# Autodesk Inventor assembly: Z-head-assembly-IKO-T1-NEMA8
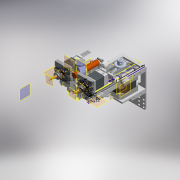
[picture p0: Inventor's stored thumbnail of the model, 180x180]
Saved by Autodesk Inventor 2016 (Build 200138000, 138)
## iProperties
Created: 2015-05-08
Part Number: Z-head-assembly-IKO-T1-NEMA8
Document SubType Name: Assembly
Designer: ax
Mass: 653.738 g
Surface Area: 1248.62 cm^2
Volume: 178.22 cm^3
Density: 3.66816 g/cm^3
Author: ax
## Documents named in this file (34)
- C:\Users\as\Documents\Inventor\mintplacer-export\Z-head-assembly-IKO-T1-NEMA8.iam
- C:\Users\as\Documents\Inventor\mintplacer-export\Z-head-baseplate-IKO.ipt
- C:\Users\as\Documents\Inventor\mintplacer-export\BSPG15_60__40_.iam
- C:\Users\as\Documents\Inventor\mintplacer-export\C-head-base.ipt
- C:\Users\as\Documents\Inventor\mintplacer-export\C-head-side.ipt
- C:\Users\as\Documents\Inventor\mintplacer-export\GT2_20tooth.ipt
- C:\Users\as\Documents\Inventor\mintplacer-export\GT2-belt-2MR-200-06.ipt
- C:\Users\as\Documents\Inventor\mintplacer-export\HTD-5M-belt-clamp.ipt
- C:\Users\as\Documents\Inventor\mintplacer-export\GT2 belt clamp.ipt
- C:\Users\as\Documents\Inventor\mintplacer-export\nozzle-assembly.iam
- C:\Users\as\Documents\Inventor\mintplacer-export\Nanotec-ST4118S1404.iam
- C:\Users\as\Documents\Inventor\mintplacer-export\c-head-flange.ipt
- C:\Users\as\Documents\Inventor\mintplacer-export\Z-head-assembly-IKO-T1\Design Accelerator\Bolted Connection3.iam
- C:\Users\as\Documents\Inventor\mintplacer-export\Z-head-assembly-IKO-T1\Design Accelerator\Bolted Connection4.iam
- C:\Users\as\Documents\Inventor\mintplacer-export\Z-head-assembly-IKO-T1\Design Accelerator\Bolted Connection5.iam
- C:\Users\as\Documents\Inventor\mintplacer-export\Z-head-assembly-IKO-T1\Design Accelerator\Bolted Connection6.iam
- C:\Users\as\Documents\Inventor\mintplacer-export\Z-head-assembly-IKO-T1\Design Accelerator\Bolted Connection7.iam
- C:\Users\as\Documents\Inventor\mintplacer-export\small-tact-switch.ipt
- C:\Users\as\Documents\Inventor\mintplacer-export\Z-head-assembly-IKO-T1\Design Accelerator\Bolted Connection8.iam
- C:\Users\as\Documents\Inventor\mintplacer-export\Z-head-assembly-IKO-T1\Design Accelerator\Bolted Connection9.iam
- C:\Users\as\Documents\Inventor\mintplacer-export\Z-head-assembly-IKO-T1\Design Accelerator\Bolted Connection10.iam
- C:\Users\as\Documents\Inventor\mintplacer-export\Z-head-assembly-IKO-T1\Design Accelerator\Bolted Connection11.iam
- C:\Users\as\Documents\Inventor\Content Center Files\R2016\en-US\ISO 4762(1)\DIN EN ISO 4762 - M3 x 12.ipt
- C:\Users\as\Documents\Inventor\mintplacer-export\render\cam-flying.iam
- C:\Users\as\Documents\Inventor\mintplacer-export\Z-head-assembly-IKO-T1\Design Accelerator\Bolted Connection13.iam
- C:\Users\as\Documents\Inventor\mintplacer-export\Z-head-assembly-IKO-T1\Design Accelerator\Bolted Connection14.iam
- C:\Users\as\Documents\Inventor\mintplacer-export\render\Z-head-sideplate.ipt
- C:\Users\as\Documents\Inventor\mintplacer-export\Z-head-topplate.ipt
- C:\Users\as\Documents\Inventor\mintplacer-export\render\Z-head-beltmount.ipt
- C:\Users\as\Documents\Inventor\mintplacer-export\Z-head-assembly-IKO-T1\Design Accelerator\Bolted Connection15.iam
- C:\Users\as\Documents\Inventor\mintplacer-export\Z-head-assembly-IKO-T1\Design Accelerator\Bolted Connection16.iam
- C:\Users\as\Documents\Inventor\mintplacer-export\Z-head-assembly-IKO-T1\Design Accelerator\Bolted Connection17.iam
- C:\Users\as\Documents\Inventor\mintplacer-export\Z-head-assembly-IKO-T1\Design Accelerator\Bolted Connection18.iam
- C:\Users\as\Documents\Inventor\mintplacer-export\Nanotec-NEMA8-st2018s0604\st2018s0604.iam
## Components (69 placed, 19 different names)
1. Z-head-baseplate-IKO:1 — Mate:1, Flush:1, Flush:7, Mate:5, Mate:10, Mate:39, Mate:40, Mate:41, Mate:70, Mate:71, Mate:74, Mate:76, Mate:110, Flush:31, Mate:111, Mate:112, Mate:116, Angle:1, Mate:118, Flush:36, Flush:37, Flush:38, Mate:121, Mate:133, Mate:135, Flush:43, Flush:44
2. HTD-5M-belt-clamp:1 — Mate:131, Flush:42
3. Nanotec-ST4118S1404:2 [sub-assembly] — Mate:5, Mate:10, Cylindrical:1, Mate:72, Mate:73, Mate:75, Flush:33, Mate:117
4. GT2_20tooth:1 — Mate:4, Cylindrical:1
5. BSPG15_60__40_:1 [sub-assembly] — Mate:1, Flush:1, Flush:3, Mate:11, Flush:19, Flush:20, Mate:84, Mate:86, Mate:122, Flush:44
6. c-head-flange:1 — Flush:14, Flush:15, Mate:11, Mate:12, Flush:17, Flush:19, Mate:32, Mate:33, Mate:34, Flush:20, Mate:83, Mate:85, Mate:87, Mate:88, Mate:130
7. C-head-base:1 — Flush:3, Flush:13, Flush:14, Flush:15, Flush:18, Mate:17, Mate:78, Mate:142, Mate:143
8. C-head-side:1 — Mate:7, Flush:11, Flush:13, Mate:12, Flush:17, Flush:18, Mate:17, Mate:77, Flush:34, Mate:129
9. st2018s0604:1 [sub-assembly] — Mate:142, Mate:143, Mate:144
10. nozzle-assembly:1 [sub-assembly] — Mate:144
11. GT2 belt clamp:1 — Mate:7, Flush:11, Flush:34, Mate:127, Mate:128
12. Bolted Connection:3 [sub-assembly] — Mate:77, Mate:78
13. Bolted Connection:4 [sub-assembly] — Mate:129, Mate:130
14. Bolted Connection:5 [sub-assembly] — Mate:127, Mate:128
15. Bolted Connection:6 [sub-assembly] — Mate:83, Mate:84
16. Bolted Connection:7 [sub-assembly] — Mate:85, Mate:86
17. small-tact-switch:1 — Mate:32, Mate:33, Mate:34, Mate:89, Mate:90
18. Bolted Connection:8 [sub-assembly] — Mate:87, Mate:88
19. small-tact-switch:2 — Mate:123, Mate:124
20. small-tact-switch:3 — Mate:39, Mate:40, Mate:41, Mate:125, Mate:126
21. Bolted Connection:9 [sub-assembly] — Mate:89, Mate:90
22. Bolted Connection:10 [sub-assembly] — Mate:125, Mate:126
23. Bolted Connection:12 [sub-assembly] — Mate:123, Mate:124
24. DIN EN ISO 4762 M3 x 12:1 — Mate:70, Mate:117
25. DIN EN ISO 4762 M3 x 12:2 — Mate:71, Mate:72
26. DIN EN ISO 4762 M3 x 12:3 — Mate:74, Mate:75
27. DIN EN ISO 4762 M3 x 12:4 — Mate:73, Mate:76
28. cam-flying:1 [sub-assembly] — Mate:110, Flush:31, Mate:111, Mate:113
29. Bolted Connection:13 [sub-assembly] — Mate:112, Mate:113
30. Bolted Connection:14 [sub-assembly] — Mate:121, Mate:122
31. Z-head-sideplate:1 — Mate:119, Flush:39, Flush:40, Mate:120, Mate:134, Mate:138
32. Z-head-topplate:1 — Flush:36, Flush:37, Flush:38, Mate:119, Flush:39, Flush:40, Flush:41, Mate:132, Mate:140
33. Z-head-beltmount:1 — Flush:41, Mate:120, Mate:131, Flush:42, Flush:43, Mate:139, Mate:141
34. Bolted Connection:15 [sub-assembly] — Mate:132, Mate:133
35. Bolted Connection:16 [sub-assembly] — Mate:134, Mate:135
36. Bolted Connection:17 [sub-assembly] — Mate:140, Mate:141
37. Bolted Connection:18 [sub-assembly] — Mate:138, Mate:139
38. BSPG15_60__40_:2 [sub-assembly] — Flush:45, Flush:50, Flush:51, Mate:148, Mate:153, Mate:155, Mate:162
39. C-head-base:2 — Flush:45, Flush:46, Mate:145, Flush:47, Flush:53, Flush:54, Mate:149, Mate:164, Mate:165
40. C-head-side:2 — Flush:46, Mate:145, Flush:47, Mate:146, Flush:48, Flush:49, Flush:52, Mate:147, Flush:55, Flush:56
41. GT2 belt clamp:2 — Mate:146, Flush:48, Flush:49, Mate:151, Mate:152
42. nozzle-assembly:2 [sub-assembly] — Mate:163
43. c-head-flange:2 — Flush:50, Flush:51, Flush:52, Mate:147, Mate:148, Flush:53, Flush:54, Mate:150, Mate:154, Mate:156, Mate:157, Mate:158, Flush:57, Mate:159, Mate:160
44. Bolted Connection:19 [sub-assembly] — Mate:149, Flush:55
45. Bolted Connection:20 [sub-assembly] — Mate:150, Flush:56
46. Bolted Connection:21 [sub-assembly] — Mate:151, Mate:152
47. Bolted Connection:22 [sub-assembly] — Mate:153, Mate:154
48. Bolted Connection:23 [sub-assembly] — Mate:155, Mate:156
49. small-tact-switch:4 — Mate:157, Mate:158, Flush:57, Mate:161, Flush:58
50. Bolted Connection:24 [sub-assembly] — Mate:159, Mate:160
51. Bolted Connection:25 [sub-assembly] — Mate:161, Flush:58
52. Bolted Connection:26 [sub-assembly] — Mate:162
53. st2018s0604:2 [sub-assembly] — Mate:163, Mate:164, Mate:165
54. GT2-belt-2MR-200-06:1 — Mate:4, Mate:118
55. GT2-belt-2MR-200-06:2
56. GT2-belt-2MR-200-06:3
57. GT2-belt-2MR-200-06:4
58. GT2-belt-2MR-200-06:5
59. GT2-belt-2MR-200-06:6
60. GT2-belt-2MR-200-06:7
61. GT2-belt-2MR-200-06:8
62. GT2-belt-2MR-200-06:9
63. GT2-belt-2MR-200-06:10
64. GT2-belt-2MR-200-06:11
65. GT2-belt-2MR-200-06:12
66. GT2-belt-2MR-200-06:13
67. GT2-belt-2MR-200-06:14
68. GT2-belt-2MR-200-06:15
69. GT2-belt-2MR-200-06:16
## Component patterns: (8 elements, first: GT2-belt-2MR-200-06:1), (8 elements, first: GT2-belt-2MR-200-06:9)
## Relationships (124: Mate 83, Flush 39, CylindricalJoint 1, Angle 1)
- Mate:1: Z-head-baseplate-IKO:1 ↔ BSPG15_60__40_:1
- Flush:1: Z-head-baseplate-IKO:1 ↔ BSPG15_60__40_:1
- Flush:3: BSPG15_60__40_:1 ↔ C-head-base:1
- Mate:4 (1 mm): GT2_20tooth:1 ↔ GT2-belt-2MR-200-06:1
- Flush:7 (-6.3662 mm): Z-head-baseplate-IKO:1
- Mate:5 (-21 mm): Z-head-baseplate-IKO:1 ↔ Nanotec-ST4118S1404:2
- Flush:8 (-1.15 mm)
- Mate:7: C-head-side:1 ↔ GT2 belt clamp:1
- Flush:11: C-head-side:1 ↔ GT2 belt clamp:1
- Flush:13: C-head-base:1 ↔ C-head-side:1
- Mate:10: Z-head-baseplate-IKO:1 ↔ Nanotec-ST4118S1404:2
- Cylindrical:1: Nanotec-ST4118S1404:2 ↔ GT2_20tooth:1
- Flush:14: c-head-flange:1 ↔ C-head-base:1
- Flush:15: c-head-flange:1 ↔ C-head-base:1
- Mate:11: BSPG15_60__40_:1 ↔ c-head-flange:1
- Mate:12: c-head-flange:1 ↔ C-head-side:1
- Flush:17: c-head-flange:1 ↔ C-head-side:1
- Flush:18: C-head-base:1 ↔ C-head-side:1
- Flush:19: BSPG15_60__40_:1 ↔ c-head-flange:1
- Mate:17: C-head-base:1 ↔ C-head-side:1
- Mate:32: c-head-flange:1 ↔ small-tact-switch:1
- Mate:33: c-head-flange:1 ↔ small-tact-switch:1
- Mate:34: c-head-flange:1 ↔ small-tact-switch:1
- Flush:20: BSPG15_60__40_:1 ↔ c-head-flange:1
- Mate:39: Z-head-baseplate-IKO:1 ↔ small-tact-switch:3
- Mate:40: Z-head-baseplate-IKO:1 ↔ small-tact-switch:3
- Mate:41: Z-head-baseplate-IKO:1 ↔ small-tact-switch:3
- Mate:70: Z-head-baseplate-IKO:1 ↔ DIN EN ISO 4762 M3 x 12:1
- Mate:71: Z-head-baseplate-IKO:1 ↔ DIN EN ISO 4762 M3 x 12:2
- Mate:72: Nanotec-ST4118S1404:2 ↔ DIN EN ISO 4762 M3 x 12:2
- Mate:73: Nanotec-ST4118S1404:2 ↔ DIN EN ISO 4762 M3 x 12:4
- Mate:74: Z-head-baseplate-IKO:1 ↔ DIN EN ISO 4762 M3 x 12:3
- Mate:75: Nanotec-ST4118S1404:2 ↔ DIN EN ISO 4762 M3 x 12:3
- Mate:76: Z-head-baseplate-IKO:1 ↔ DIN EN ISO 4762 M3 x 12:4
- Mate:77: C-head-side:1 ↔ Bolted Connection:3
- Mate:78: C-head-base:1 ↔ Bolted Connection:3
- Mate:83: c-head-flange:1 ↔ Bolted Connection:6
- Mate:84: BSPG15_60__40_:1 ↔ Bolted Connection:6
- Mate:85: c-head-flange:1 ↔ Bolted Connection:7
- Mate:86: BSPG15_60__40_:1 ↔ Bolted Connection:7
- Mate:87: c-head-flange:1 ↔ Bolted Connection:8
- Mate:88: c-head-flange:1 ↔ Bolted Connection:8
- Mate:89: small-tact-switch:1 ↔ Bolted Connection:9
- Mate:90: small-tact-switch:1 ↔ Bolted Connection:9
- Mate:110: Z-head-baseplate-IKO:1 ↔ cam-flying:1
- Flush:31: Z-head-baseplate-IKO:1 ↔ cam-flying:1
- Mate:111: Z-head-baseplate-IKO:1 ↔ cam-flying:1
- Mate:112: Z-head-baseplate-IKO:1 ↔ Bolted Connection:13
- Mate:113: cam-flying:1 ↔ Bolted Connection:13
- Mate:116: Z-head-baseplate-IKO:1
- Angle:1 (0 deg): Z-head-baseplate-IKO:1
- Flush:32 (-79 mm)
- Flush:33 (-21 mm): Nanotec-ST4118S1404:2
- Mate:117: Nanotec-ST4118S1404:2 ↔ DIN EN ISO 4762 M3 x 12:1
- Flush:34: C-head-side:1 ↔ GT2 belt clamp:1
- Mate:118 (-7 mm): Z-head-baseplate-IKO:1 ↔ GT2-belt-2MR-200-06:1
- Flush:36: Z-head-baseplate-IKO:1 ↔ Z-head-topplate:1
- Flush:37: Z-head-baseplate-IKO:1 ↔ Z-head-topplate:1
- Flush:38: Z-head-baseplate-IKO:1 ↔ Z-head-topplate:1
- Mate:119: Z-head-sideplate:1 ↔ Z-head-topplate:1
- Flush:39: Z-head-sideplate:1 ↔ Z-head-topplate:1
- Flush:40: Z-head-sideplate:1 ↔ Z-head-topplate:1
- Flush:41: Z-head-topplate:1 ↔ Z-head-beltmount:1
- Mate:120: Z-head-sideplate:1 ↔ Z-head-beltmount:1
- Mate:121: Z-head-baseplate-IKO:1 ↔ Bolted Connection:14
- Mate:122: BSPG15_60__40_:1 ↔ Bolted Connection:14
- Mate:123: small-tact-switch:2 ↔ Bolted Connection:12
- Mate:124: small-tact-switch:2 ↔ Bolted Connection:12
- Mate:125: small-tact-switch:3 ↔ Bolted Connection:10
- Mate:126: small-tact-switch:3 ↔ Bolted Connection:10
- Mate:127: GT2 belt clamp:1 ↔ Bolted Connection:5
- Mate:128: GT2 belt clamp:1 ↔ Bolted Connection:5
- Mate:129: C-head-side:1 ↔ Bolted Connection:4
- Mate:130: c-head-flange:1 ↔ Bolted Connection:4
- Mate:131: HTD-5M-belt-clamp:1 ↔ Z-head-beltmount:1
- Flush:42: HTD-5M-belt-clamp:1 ↔ Z-head-beltmount:1
- Mate:132: Z-head-topplate:1 ↔ Bolted Connection:15
- Mate:133: Z-head-baseplate-IKO:1 ↔ Bolted Connection:15
- Mate:134: Z-head-sideplate:1 ↔ Bolted Connection:16
- Mate:135: Z-head-baseplate-IKO:1 ↔ Bolted Connection:16
- Flush:43 (-35 mm): Z-head-baseplate-IKO:1 ↔ Z-head-beltmount:1
- Mate:138: Z-head-sideplate:1 ↔ Bolted Connection:18
- Mate:139: Z-head-beltmount:1 ↔ Bolted Connection:18
- Mate:140: Z-head-topplate:1 ↔ Bolted Connection:17
- Mate:141: Z-head-beltmount:1 ↔ Bolted Connection:17
- Mate:142: C-head-base:1 ↔ st2018s0604:1
- Mate:143: C-head-base:1 ↔ st2018s0604:1
- Flush:44 (2.5 mm): Z-head-baseplate-IKO:1 ↔ BSPG15_60__40_:1
- Mate:144: st2018s0604:1 ↔ nozzle-assembly:1
- Flush:45: BSPG15_60__40_:2 ↔ C-head-base:2
- Flush:46: C-head-base:2 ↔ C-head-side:2
- Mate:145: C-head-base:2 ↔ C-head-side:2
- Flush:47: C-head-base:2 ↔ C-head-side:2
- Mate:146: C-head-side:2 ↔ GT2 belt clamp:2
- Flush:48: C-head-side:2 ↔ GT2 belt clamp:2
- Flush:49: C-head-side:2 ↔ GT2 belt clamp:2
- Flush:50: BSPG15_60__40_:2 ↔ c-head-flange:2
- Flush:51: BSPG15_60__40_:2 ↔ c-head-flange:2
- Flush:52: C-head-side:2 ↔ c-head-flange:2
- Mate:147: C-head-side:2 ↔ c-head-flange:2
- Mate:148: BSPG15_60__40_:2 ↔ c-head-flange:2
- Flush:53: C-head-base:2 ↔ c-head-flange:2
- Flush:54: C-head-base:2 ↔ c-head-flange:2
- Mate:149: C-head-base:2 ↔ Bolted Connection:19
- Flush:55: C-head-side:2 ↔ Bolted Connection:19
- Mate:150: c-head-flange:2 ↔ Bolted Connection:20
- Flush:56: C-head-side:2 ↔ Bolted Connection:20
- Mate:151: GT2 belt clamp:2 ↔ Bolted Connection:21
- Mate:152: GT2 belt clamp:2 ↔ Bolted Connection:21
- Mate:153: BSPG15_60__40_:2 ↔ Bolted Connection:22
- Mate:154: c-head-flange:2 ↔ Bolted Connection:22
- Mate:155: BSPG15_60__40_:2 ↔ Bolted Connection:23
- Mate:156: c-head-flange:2 ↔ Bolted Connection:23
- Mate:157: c-head-flange:2 ↔ small-tact-switch:4
- Mate:158: c-head-flange:2 ↔ small-tact-switch:4
- Flush:57: c-head-flange:2 ↔ small-tact-switch:4
- Mate:159: c-head-flange:2 ↔ Bolted Connection:24
- Mate:160: c-head-flange:2 ↔ Bolted Connection:24
- Mate:161: small-tact-switch:4 ↔ Bolted Connection:25
- Flush:58: small-tact-switch:4 ↔ Bolted Connection:25
- Mate:162: BSPG15_60__40_:2 ↔ Bolted Connection:26
- Mate:163: nozzle-assembly:2 ↔ st2018s0604:2
- Mate:164: C-head-base:2 ↔ st2018s0604:2
- Mate:165: C-head-base:2 ↔ st2018s0604:2
## Named parameters: pulleyTeeth = 20, cPulley = 40 mm, dPulley = 12.7324 mm, beltThickness = 1.15 mm
